# Autodesk Inventor assembly: Mould assembly
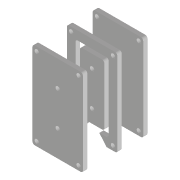
[picture p0: Inventor's stored thumbnail of the model, 180x180]
Saved by Autodesk Inventor 2020 (Build 240168000, 168)
## iProperties
Created: 2022-03-07
Part Number: Mould assembly
Document SubType Name: Assembly
Designer: ferrerx
Author: ferrerx
## Documents named in this file (4)
- C:\Users\ferrerx\Desktop\Aureliene mould\Mould assembly.iam
- C:\Users\ferrerx\Desktop\Aureliene mould\Middle external.ipt
- C:\Users\ferrerx\Desktop\Aureliene mould\Middle internal.ipt
- C:\Users\ferrerx\Desktop\Aureliene mould\Top&Bottom.ipt
## Components (4 placed, 3 different names)
1. Middle external:1 — Mate:3, Mate:4, Flush:1
2. Middle internal:1 — Mate:1, Mate:2, Flush:1
3. Top&Bottom:1 — Mate:5, Mate:6
4. Top&Bottom:2 — Mate:1, Mate:2, Mate:3, Mate:4, Mate:5, Mate:6
## Relationships (7: Mate 6, Flush 1)
- Mate:1: Middle internal:1 ↔ Top&Bottom:2
- Mate:2: Middle internal:1 ↔ Top&Bottom:2
- Mate:3: Middle external:1 ↔ Top&Bottom:2
- Mate:4: Middle external:1 ↔ Top&Bottom:2
- Mate:5: Top&Bottom:1 ↔ Top&Bottom:2
- Mate:6: Top&Bottom:1 ↔ Top&Bottom:2
- Flush:1: Middle external:1 ↔ Middle internal:1
